# Autodesk Inventor assembly: encoder_ass_MIR1
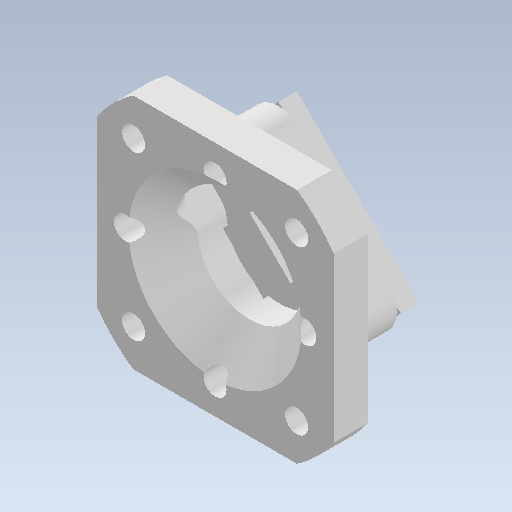
[picture p0: Inventor's stored thumbnail of the model, 512x512]
Saved by Autodesk Inventor 2020 (Build 240168000, 168)
## iProperties
Created: 2019-05-18
Part Number: encoder_ass_MIR1
Document SubType Name: Assembly
Designer: psrob
Author: psrob
## Documents named in this file (3)
- E:\projects-2\project dog gen2\hardware\encoder_ass_MIR1.iam
- E:\projects-2\project dog gen2\hardware\encoder_holder_MIR.ipt
- E:\projects-2\project dog gen2\hardware\encoder_m_MIR1.iam
## Components (2 placed, 2 different names)
1. encoder_holder_MIR:1 — Insert:2, Insert:1
2. encoder_m_MIR1:1 [sub-assembly] — Insert:2, Insert:1
## Relationships (2: Insert 2)
- Insert:2: encoder_holder_MIR:1 ↔ encoder_m_MIR1:1
- Insert:1: encoder_holder_MIR:1 ↔ encoder_m_MIR1:1
